# Autodesk Inventor assembly: cam_holder
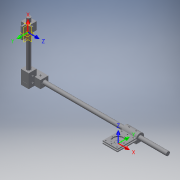
[picture p0: Inventor's stored thumbnail of the model, 180x180]
Saved by Autodesk Inventor 2019 (Build 230136000, 136)
## iProperties
Created: 2024-08-06
Part Number: cam_holder
Material: Generisch
Document SubType Name: Assembly
Designer: nic
Author: nic
## Documents named in this file (7)
- C:\Users\Nicolas Frick\Sync\OneDrive\wtm\nicol_rh8d\inventor\cam_holder.iam
- C:\Users\Nicolas Frick\Sync\OneDrive\wtm\nicol_rh8d\inventor\pipe_700.ipt
- C:\Users\Nicolas Frick\Sync\OneDrive\wtm\nicol_rh8d\inventor\pipe_300.ipt
- C:\Users\Nicolas Frick\Sync\OneDrive\wtm\nicol_rh8d\inventor\cam_holder_angle_part_aligned.iam
- C:\Users\Nicolas Frick\Sync\OneDrive\wtm\nicol_rh8d\inventor\cam_holder_end_part_aligned.iam
- C:\Users\Nicolas Frick\Sync\OneDrive\wtm\nicol_rh8d\inventor\cam_holder_wrist_part_aligned.iam
- C:\Users\Nicolas Frick\Sync\OneDrive\wtm\nicol_rh8d\inventor\cam_holder_hog_part_aligned.iam
## Components (6 placed, 6 different names)
1. pipe_700:1 — Passend:15, Passend:18, Fluchtend:7
2. pipe_300:1 — Passend:19, Fluchtend:9, Passend:20
3. cam_holder_end_part_aligned:1 [sub-assembly] — Passend:20, Z, Fluchtend:11, Passend:22, Passend:23, Fluchtend:12
4. cam_holder_wrist_part_aligned:1 [sub-assembly] — Passend:15, Passend:16, Passend:17, Theta, Fluchtend:8
5. cam_holder_angle_part_aligned:1 [sub-assembly] — Passend:18, Fluchtend:7, Fluchtend:8, Passend:19, Fluchtend:9, Z, Fluchtend:11, X
6. cam_holder_hog_part_aligned:1 [sub-assembly] — Passend:22, Passend:23, Fluchtend:12
## Relationships (16: Mate 9, Flush 7)
- Passend:15 [Mate]: pipe_700:1 ↔ cam_holder_wrist_part_aligned:1
- Passend:16 [Mate]: cam_holder_wrist_part_aligned:1
- Passend:17 [Mate]: cam_holder_wrist_part_aligned:1
- Theta [Flush]: cam_holder_wrist_part_aligned:1
- Passend:18 [Mate]: pipe_700:1 ↔ cam_holder_angle_part_aligned:1
- Fluchtend:7 [Flush]: pipe_700:1 ↔ cam_holder_angle_part_aligned:1
- Fluchtend:8 [Flush]: cam_holder_wrist_part_aligned:1 ↔ cam_holder_angle_part_aligned:1
- Passend:19 [Mate]: pipe_300:1 ↔ cam_holder_angle_part_aligned:1
- Fluchtend:9 [Flush]: pipe_300:1 ↔ cam_holder_angle_part_aligned:1
- Passend:20 [Mate]: pipe_300:1 ↔ cam_holder_end_part_aligned:1
- Z [Flush] (240 mm): cam_holder_end_part_aligned:1 ↔ cam_holder_angle_part_aligned:1
- Fluchtend:11 [Flush]: cam_holder_end_part_aligned:1 ↔ cam_holder_angle_part_aligned:1
- X [Mate] (-500 mm): cam_holder_angle_part_aligned:1
- Passend:22 [Mate]: cam_holder_end_part_aligned:1 ↔ cam_holder_hog_part_aligned:1
- Passend:23 [Mate]: cam_holder_end_part_aligned:1 ↔ cam_holder_hog_part_aligned:1
- Fluchtend:12 [Flush]: cam_holder_end_part_aligned:1 ↔ cam_holder_hog_part_aligned:1
